# Autodesk Inventor assembly: inner
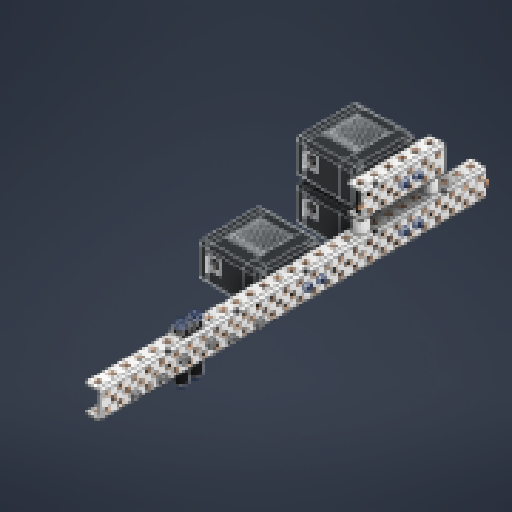
[picture p0: Inventor's stored thumbnail of the model, 512x512]
Saved by Autodesk Inventor 2024 (Build 280153000, 153)
## iProperties
Created: 2023-10-18
Part Number: inner
Document SubType Name: Assembly
Designer: Averey Ku
Author: Averey Ku
## Documents named in this file (18)
- D:\vex_robotics\hardware\cad\goated_v0.1\chassis\drivebay\inner.iam
- D:\vex_robotics\hardware\cad\VEX-CAD-Inventor-1.41\Structure\C Channel\Aluminum 1x2x1\Alu C 1x2x1x28.ipt
- D:\vex_robotics\hardware\cad\VEX-CAD-Inventor-1.41\Structure\C Channel\Aluminum 1x2x1\Alu C 1x2x1x6.ipt
- D:\vex_robotics\hardware\cad\VEX-CAD-Inventor-1.41\Structure\Standoff\Standoff .875.ipt
- D:\vex_robotics\hardware\cad\VEX-CAD-Inventor-1.41\Structure\Standoff.ipt
- D:\vex_robotics\hardware\cad\hardware\.375 OD Aluminum Spacer 0.875.ipt
- D:\vex_robotics\hardware\cad\VEX-CAD-Inventor-1.41\Electronics\Motors with Screws\SteelM-StarS.iam
- D:\vex_robotics\hardware\cad\VEX-CAD-Inventor-1.41\Electronics\Motors with Screws.iam
- D:\vex_robotics\hardware\cad\VEX-CAD-Inventor-1.41\Motion\Spacers\Spacer Nylon .500 OD\NSpacer White .500 OD x .500.ipt
- D:\vex_robotics\hardware\cad\VEX-CAD-Inventor-1.41\Motion\Spacers\Spacer Nylon .500 OD.ipt
- D:\vex_robotics\hardware\cad\VEX-CAD-Inventor-1.41\lightweight_bearing.iam
- D:\vex_robotics\hardware\cad\VEX-CAD-Inventor-1.41\Motion\Spacers\Spacer Nylon .375 OD\NSpacer .375 OD x .500.ipt
- D:\vex_robotics\hardware\cad\VEX-CAD-Inventor-1.41\Motion\Spacers\Spacer Nylon .375 OD.ipt
- D:\vex_robotics\hardware\cad\VEX-CAD-Inventor-1.41\Structure\Hardware\Nut Keps.ipt
- D:\vex_robotics\hardware\cad\goated_v0.1\chassis\drivebay\custom_parts\short_bearing.ipt
- D:\vex_robotics\hardware\cad\VEX-CAD-Inventor-1.41\Structure\Hardware\Screw Shoulder Robosource\SScrew Shoulder Smooth 2.000 x .04.ipt
- D:\vex_robotics\hardware\cad\VEX-CAD-Inventor-1.41\Structure\Hardware\Screw Shoulder Robosource.ipt
- D:\vex_robotics\hardware\cad\VEX-CAD-Inventor-1.41\Structure\Hardware\Nut Hex.ipt
## Components (24 placed, 12 different names)
1. Alu C 1x2x1x28:1 — Insert:3, Mate:1, Insert:4, Insert:6, Mate:3, Insert:7, Insert:8, Insert:9, Mate:4, Insert:10, Mate:5, Insert:11, Mate:6, Insert:12, Mate:7, Insert:13, Insert:14, Insert:15, Insert:16, Insert:17, Insert:18, Insert:19, Mate:8
2. Alu C 1x2x1x6:1 — Insert:3, Mate:1, Insert:5, Mate:2
3. Standoff .875:1
4. Standoff .875:2
5. .375 OD Aluminum Spacer 0.875:1 — Insert:4
6. SteelM-StarS:1 [sub-assembly] — Insert:5, Mate:2
7. SteelM-StarS:2 [sub-assembly] — Insert:6, Mate:3
8. NSpacer White .500 OD x .500:1 — Insert:8
9. NSpacer White .500 OD x .500:2 — Insert:7
10. SteelM-StarS:3 [sub-assembly] — Insert:9, Mate:4
11. lightweight_bearing:1 [sub-assembly] — Insert:10, Mate:5
12. lightweight_bearing:2 [sub-assembly] — Insert:11, Mate:6
13. lightweight_bearing:3 [sub-assembly] — Insert:12, Mate:7
14. NSpacer .375 OD x .500:1 — Insert:14, Insert:21
15. NSpacer .375 OD x .500:2 — Insert:13, Insert:20
16. Nut Keps:1 — Insert:18
17. Nut Keps:2 — Insert:17
18. Nut Keps:3 — Insert:16
19. Nut Keps:4 — Insert:15
20. short_bearing:1 — Insert:19, Mate:8, Insert:22, Insert:23
21. SScrew Shoulder Smooth 2.000 x .04:1 — Insert:20
22. SScrew Shoulder Smooth 2.000 x .04:2 — Insert:21
23. Nut Hex:1 — Insert:22
24. Nut Hex:2 — Insert:23
## Relationships (31: Insert 23, Mate 8)
- [Insert]: Alu C 1x2x1x6:1 ↔ Standoff .875:1
- [Insert]: Alu C 1x2x1x6:1 ↔ Standoff .875:2
- Insert:3 (12.7 mm): Alu C 1x2x1x28:1 ↔ Alu C 1x2x1x6:1
- Mate:1: Alu C 1x2x1x28:1 ↔ Alu C 1x2x1x6:1
- Insert:4: Alu C 1x2x1x28:1 ↔ .375 OD Aluminum Spacer 0.875:1
- Insert:5: Alu C 1x2x1x6:1 ↔ SteelM-StarS:1
- Mate:2: Alu C 1x2x1x6:1 ↔ SteelM-StarS:1
- Insert:6: Alu C 1x2x1x28:1 ↔ SteelM-StarS:2
- Mate:3: Alu C 1x2x1x28:1 ↔ SteelM-StarS:2
- Insert:7: Alu C 1x2x1x28:1 ↔ NSpacer White .500 OD x .500:2
- Insert:8: Alu C 1x2x1x28:1 ↔ NSpacer White .500 OD x .500:1
- Insert:9: Alu C 1x2x1x28:1 ↔ SteelM-StarS:3
- Mate:4: Alu C 1x2x1x28:1 ↔ SteelM-StarS:3
- Insert:10: Alu C 1x2x1x28:1 ↔ lightweight_bearing:1
- Mate:5: Alu C 1x2x1x28:1 ↔ lightweight_bearing:1
- Insert:11: Alu C 1x2x1x28:1 ↔ lightweight_bearing:2
- Mate:6: Alu C 1x2x1x28:1 ↔ lightweight_bearing:2
- Insert:12: Alu C 1x2x1x28:1 ↔ lightweight_bearing:3
- Mate:7: Alu C 1x2x1x28:1 ↔ lightweight_bearing:3
- Insert:13: Alu C 1x2x1x28:1 ↔ NSpacer .375 OD x .500:2
- Insert:14: Alu C 1x2x1x28:1 ↔ NSpacer .375 OD x .500:1
- Insert:15: Alu C 1x2x1x28:1 ↔ Nut Keps:4
- Insert:16: Alu C 1x2x1x28:1 ↔ Nut Keps:3
- Insert:17: Alu C 1x2x1x28:1 ↔ Nut Keps:2
- Insert:18: Alu C 1x2x1x28:1 ↔ Nut Keps:1
- Insert:19: Alu C 1x2x1x28:1 ↔ short_bearing:1
- Mate:8: Alu C 1x2x1x28:1 ↔ short_bearing:1
- Insert:20 (1.5875 mm): NSpacer .375 OD x .500:2 ↔ SScrew Shoulder Smooth 2.000 x .04:1
- Insert:21 (1.5875 mm): NSpacer .375 OD x .500:1 ↔ SScrew Shoulder Smooth 2.000 x .04:2
- Insert:22: short_bearing:1 ↔ Nut Hex:1
- Insert:23: short_bearing:1 ↔ Nut Hex:2
